# Autodesk Inventor assembly: blob_all
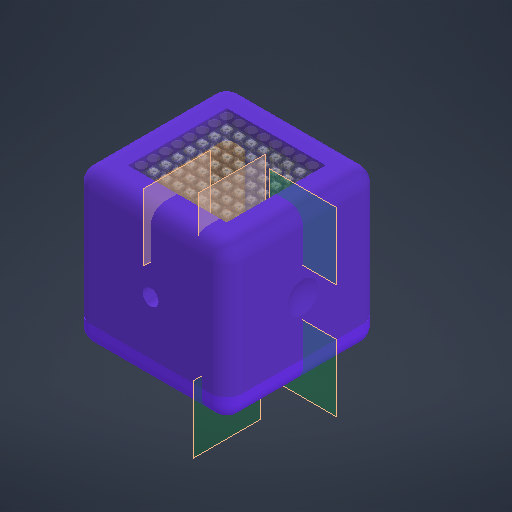
[picture p0: Inventor's stored thumbnail of the model, 512x512]
Saved by Autodesk Inventor 2025.2 (Build 292293000, 293)
## iProperties
Created: 2025-06-28
Part Number: blob_all
Document SubType Name: Assembly
Designer: micyg
Author: micyg
## Documents named in this file (5)
- D:\Projects\VirtualPets\VirtualBlob\Mechanical\blob_all.iam
- D:\Projects\VirtualPets\VirtualBlob\Mechanical\case1.ipt
- D:\Projects\VirtualPets\VirtualBlob\Mechanical\case2.ipt
- D:\Projects\VirtualPets\VirtualBlob\Mechanical\battery.ipt
- D:\Projects\VirtualPets\VirtualBlob\Mechanical\matrix\matrix_V2.iam
## Components (4 placed, 4 different names)
1. case1:1 — Mate:1, Mate:2, Mate:3, Mate:5, Mate:7, Mate:8, Mate:9, Mate:10
2. case2:1 — Mate:3, Mate:9, Mate:10
3. battery:1 — Mate:1, Mate:2
4. matrix_V2:1 [sub-assembly] — Mate:5, Mate:7, Mate:8
## Relationships (8: Mate 8)
- Mate:1: case1:1 ↔ battery:1
- Mate:2: case1:1 ↔ battery:1
- Mate:3: case1:1 ↔ case2:1
- Mate:5: case1:1 ↔ matrix_V2:1
- Mate:7 (0.25 mm): case1:1 ↔ matrix_V2:1
- Mate:8 (0.25 mm): case1:1 ↔ matrix_V2:1
- Mate:9: case1:1 ↔ case2:1
- Mate:10: case1:1 ↔ case2:1
